# Autodesk Inventor assembly: Sensor_module_envBoard
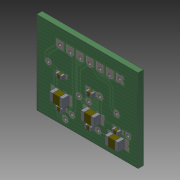
[picture p0: Inventor's stored thumbnail of the model, 180x180]
Saved by Autodesk Inventor 2013 (Build 170138000, 138)
## iProperties
Created: 2015-06-30
Part Number: Sensor_module_envBoard
Document SubType Name: Assembly
Designer: terg
Author: terg
## Documents named in this file (11)
- C:\Users\terg\Projects\ModularElectronics\3D_models\Sensor_module\Sensor_module_envBoard.iam
- C:\Users\terg\Projects\ModularElectronics\3D_models\Sensor_module\Sensor_module_envBoard_PCB.ipt
- C:\Users\terg\Projects\ModularElectronics\3D_models\Components\0402_cap.ipt
- C:\Users\terg\Projects\ModularElectronics\3D_models\Components\0805_cap.ipt
- C:\Users\terg\Projects\ModularElectronics\3D_models\Sensor_module\BMP180.ipt
- C:\Users\terg\Projects\ModularElectronics\3D_models\Sensor_module\Si7021.ipt
- C:\Users\terg\Projects\ModularElectronics\3D_models\Sensor_module\Si1143.ipt
- C:\Users\terg\Projects\ModularElectronics\3D_models\Sensor_module\TMP006.ipt
- C:\Users\terg\Projects\ModularElectronics\3D_models\Sensor_module\BH1745NUC.ipt
- C:\Users\terg\Projects\ModularElectronics\3D_models\Components\0402_res.ipt
- C:\Users\terg\Projects\ModularElectronics\3D_models\Components\0603_led.ipt
## Components (23 placed, 10 different names)
1. Sensor_module_envBoard_PCB:1 — Zestawiający:1, Zestawiający:2, Zestawiający:3, Zestawiający:4, Zestawiający:5, Zestawiający:6, Zestawiający:7, Zestawiający:8, Równoległy:1, Równoległy:2, Równoległy:3, Równoległy:4, Równoległy:5, Równoległy:6, Równoległy:7, Równoległy:8, Równoległy:9, Równoległy:10, Równoległy:11, Równoległy:12, Równoległy:13, Równoległy:14, Równoległy:15, Równoległy:16, Równoległy:17, Zestawiający:9, Równoległy:18, Zestawiający:10, Równoległy:19, Równoległy:20, Zestawiający:11, Równoległy:21, Równoległy:22, Zestawiający:12, Równoległy:23, Równoległy:24, Zestawiający:13, Równoległy:25, Równoległy:26, Zestawiający:14, Zestawiający:15, Zestawiający:16, Zestawiający:17, Zestawiający:18, Równoległy:27, Równoległy:28, Równoległy:29, Równoległy:30, Równoległy:31, Równoległy:32, Równoległy:33, Równoległy:34, Równoległy:35, Równoległy:36, Zestawiający:19, Zestawiający:20, Zestawiający:21, Zestawiający:22, Równoległy:37, Równoległy:38, Równoległy:39, Równoległy:40, Równoległy:41, Równoległy:42, Równoległy:43, Równoległy:44
2. 0402_cap:1 — Zestawiający:3, Równoległy:15, Równoległy:16
3. 0402_cap:2 — Zestawiający:5, Równoległy:8, Równoległy:12
4. 0402_cap:3 — Zestawiający:2, Równoległy:6, Równoległy:9
5. 0402_cap:4 — Zestawiający:4, Równoległy:3, Równoległy:14
6. 0402_cap:5 — Zestawiający:1, Równoległy:5, Równoległy:13
7. 0805_cap:1 — Zestawiający:8, Równoległy:7, Równoległy:11
8. 0805_cap:2 — Zestawiający:7, Równoległy:4, Równoległy:10
9. 0805_cap:3 — Zestawiający:6, Równoległy:1, Równoległy:2
10. BMP180:1 — Równoległy:17, Zestawiający:9, Równoległy:18
11. Si7021:1 — Zestawiający:10, Równoległy:19, Równoległy:20
12. Si1143:1 — Zestawiający:11, Równoległy:21, Równoległy:22
13. TMP006:1 — Zestawiający:12, Równoległy:23, Równoległy:24
14. BH1745NUC:1 — Zestawiający:13, Równoległy:25, Równoległy:26
15. 0402_res:1 — Zestawiający:14, Równoległy:27, Równoległy:36
16. 0402_res:2 — Zestawiający:15, Równoległy:28, Równoległy:35
17. 0402_res:3 — Zestawiający:16, Równoległy:29, Równoległy:34
18. 0402_res:4 — Zestawiający:17, Równoległy:30, Równoległy:33
19. 0402_res:5 — Zestawiający:18, Równoległy:31, Równoległy:32
20. 0603_led:1 — Zestawiający:19, Równoległy:37, Równoległy:41
21. 0603_led:2 — Zestawiający:20, Równoległy:39, Równoległy:43
22. 0603_led:3 — Zestawiający:21, Równoległy:40, Równoległy:44
23. 0603_led:4 — Zestawiający:22, Równoległy:38, Równoległy:42
## Relationships (66: Flush 44, Mate 22)
- Zestawiający:1 [Mate]: Sensor_module_envBoard_PCB:1 ↔ 0402_cap:5
- Zestawiający:2 [Mate]: Sensor_module_envBoard_PCB:1 ↔ 0402_cap:3
- Zestawiający:3 [Mate]: Sensor_module_envBoard_PCB:1 ↔ 0402_cap:1
- Zestawiający:4 [Mate]: Sensor_module_envBoard_PCB:1 ↔ 0402_cap:4
- Zestawiający:5 [Mate]: Sensor_module_envBoard_PCB:1 ↔ 0402_cap:2
- Zestawiający:6 [Mate]: Sensor_module_envBoard_PCB:1 ↔ 0805_cap:3
- Zestawiający:7 [Mate]: Sensor_module_envBoard_PCB:1 ↔ 0805_cap:2
- Zestawiający:8 [Mate]: Sensor_module_envBoard_PCB:1 ↔ 0805_cap:1
- Równoległy:1 [Flush] (8.114 mm): Sensor_module_envBoard_PCB:1 ↔ 0805_cap:3
- Równoległy:2 [Flush] (2.87 mm): Sensor_module_envBoard_PCB:1 ↔ 0805_cap:3
- Równoległy:3 [Flush] (3.295 mm): Sensor_module_envBoard_PCB:1 ↔ 0402_cap:4
- Równoległy:4 [Flush] (7.578 mm): Sensor_module_envBoard_PCB:1 ↔ 0805_cap:2
- Równoległy:5 [Flush] (3.261 mm): Sensor_module_envBoard_PCB:1 ↔ 0402_cap:5
- Równoległy:6 [Flush] (7.808 mm): Sensor_module_envBoard_PCB:1 ↔ 0402_cap:3
- Równoległy:7 [Flush] (11.202 mm): Sensor_module_envBoard_PCB:1 ↔ 0805_cap:1
- Równoległy:8 [Flush] (11.758 mm): Sensor_module_envBoard_PCB:1 ↔ 0402_cap:2
- Równoległy:9 [Flush] (5.753 mm): Sensor_module_envBoard_PCB:1 ↔ 0402_cap:3
- Równoległy:10 [Flush] (8.23 mm): Sensor_module_envBoard_PCB:1 ↔ 0805_cap:2
- Równoległy:11 [Flush] (9.642 mm): Sensor_module_envBoard_PCB:1 ↔ 0805_cap:1
- Równoległy:12 [Flush] (8.751 mm): Sensor_module_envBoard_PCB:1 ↔ 0402_cap:2
- Równoległy:13 [Flush] (5.719 mm): Sensor_module_envBoard_PCB:1 ↔ 0402_cap:5
- Równoległy:14 [Flush] (1.973 mm): Sensor_module_envBoard_PCB:1 ↔ 0402_cap:4
- Równoległy:15 [Flush] (1.759 mm): Sensor_module_envBoard_PCB:1 ↔ 0402_cap:1
- Równoległy:16 [Flush] (7.688 mm): Sensor_module_envBoard_PCB:1 ↔ 0402_cap:1
- Równoległy:17 [Flush] (1.58 mm): Sensor_module_envBoard_PCB:1 ↔ BMP180:1
- Zestawiający:9 [Mate]: Sensor_module_envBoard_PCB:1 ↔ BMP180:1
- Równoległy:18 [Flush] (5.571 mm): Sensor_module_envBoard_PCB:1 ↔ BMP180:1
- Zestawiający:10 [Mate]: Sensor_module_envBoard_PCB:1 ↔ Si7021:1
- Równoległy:19 [Flush] (7.5 mm): Sensor_module_envBoard_PCB:1 ↔ Si7021:1
- Równoległy:20 [Flush] (1.49 mm): Sensor_module_envBoard_PCB:1 ↔ Si7021:1
- Zestawiający:11 [Mate]: Sensor_module_envBoard_PCB:1 ↔ Si1143:1
- Równoległy:21 [Flush] (2.518 mm): Sensor_module_envBoard_PCB:1 ↔ Si1143:1
- Równoległy:22 [Flush] (2.45 mm): Sensor_module_envBoard_PCB:1 ↔ Si1143:1
- Zestawiający:12 [Mate]: Sensor_module_envBoard_PCB:1 ↔ TMP006:1
- Równoległy:23 [Flush] (4.033 mm): Sensor_module_envBoard_PCB:1 ↔ TMP006:1
- Równoległy:24 [Flush] (6.763 mm): Sensor_module_envBoard_PCB:1 ↔ TMP006:1
- Zestawiający:13 [Mate]: Sensor_module_envBoard_PCB:1 ↔ BH1745NUC:1
- Równoległy:25 [Flush] (2.8 mm): Sensor_module_envBoard_PCB:1 ↔ BH1745NUC:1
- Równoległy:26 [Flush] (3.701 mm): Sensor_module_envBoard_PCB:1 ↔ BH1745NUC:1
- Zestawiający:14 [Mate]: Sensor_module_envBoard_PCB:1 ↔ 0402_res:1
- Zestawiający:15 [Mate]: Sensor_module_envBoard_PCB:1 ↔ 0402_res:2
- Zestawiający:16 [Mate]: Sensor_module_envBoard_PCB:1 ↔ 0402_res:3
- Zestawiający:17 [Mate]: Sensor_module_envBoard_PCB:1 ↔ 0402_res:4
- Zestawiający:18 [Mate]: Sensor_module_envBoard_PCB:1 ↔ 0402_res:5
- Równoległy:27 [Flush] (1.405 mm): Sensor_module_envBoard_PCB:1 ↔ 0402_res:1
- Równoległy:28 [Flush] (1.424 mm): Sensor_module_envBoard_PCB:1 ↔ 0402_res:2
- Równoległy:29 [Flush] (1.467 mm): Sensor_module_envBoard_PCB:1 ↔ 0402_res:3
- Równoległy:30 [Flush] (1.391 mm): Sensor_module_envBoard_PCB:1 ↔ 0402_res:4
- Równoległy:31 [Flush] (1.408 mm): Sensor_module_envBoard_PCB:1 ↔ 0402_res:5
- Równoległy:32 [Flush] (4.02 mm): Sensor_module_envBoard_PCB:1 ↔ 0402_res:5
- Równoległy:33 [Flush] (5.412 mm): Sensor_module_envBoard_PCB:1 ↔ 0402_res:4
- Równoległy:34 [Flush] (7.01 mm): Sensor_module_envBoard_PCB:1 ↔ 0402_res:3
- Równoległy:35 [Flush] (8.42 mm): Sensor_module_envBoard_PCB:1 ↔ 0402_res:2
- Równoległy:36 [Flush] (9.906 mm): Sensor_module_envBoard_PCB:1 ↔ 0402_res:1
- Zestawiający:19 [Mate]: Sensor_module_envBoard_PCB:1 ↔ 0603_led:1
- Zestawiający:20 [Mate]: Sensor_module_envBoard_PCB:1 ↔ 0603_led:2
- Zestawiający:21 [Mate]: Sensor_module_envBoard_PCB:1 ↔ 0603_led:3
- Zestawiający:22 [Mate]: Sensor_module_envBoard_PCB:1 ↔ 0603_led:4
- Równoległy:37 [Flush] (0.612 mm): Sensor_module_envBoard_PCB:1 ↔ 0603_led:1
- Równoległy:38 [Flush] (2.849 mm): Sensor_module_envBoard_PCB:1 ↔ 0603_led:4
- Równoległy:39 [Flush] (5.442 mm): Sensor_module_envBoard_PCB:1 ↔ 0603_led:2
- Równoległy:40 [Flush] (7.269 mm): Sensor_module_envBoard_PCB:1 ↔ 0603_led:3
- Równoległy:41 [Flush] (2.689 mm): Sensor_module_envBoard_PCB:1 ↔ 0603_led:1
- Równoległy:42 [Flush] (0.793 mm): Sensor_module_envBoard_PCB:1 ↔ 0603_led:4
- Równoległy:43 [Flush] (2.662 mm): Sensor_module_envBoard_PCB:1 ↔ 0603_led:2
- Równoległy:44 [Flush] (1.366 mm): Sensor_module_envBoard_PCB:1 ↔ 0603_led:3
